# Autodesk Inventor assembly: ASY MSC 900.5 base frame
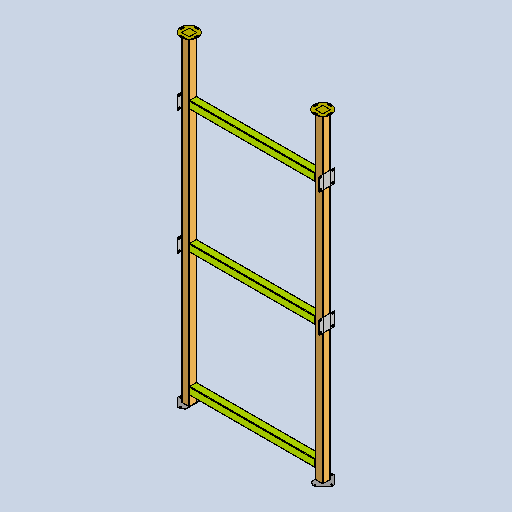
[picture p0: Inventor's stored thumbnail of the model, 512x512]
Saved by Autodesk Inventor 2025 (Build 290162010, 162A)
## iProperties
_SolveAssemblyDoc: Frame Generator Solve Assembly
_Version: 25.0.0
Created: 2024-06-27
Part Number: ASY MSC 900.5 base frame
Document SubType Name: Assembly
Designer: admin
Stock Number: ASY МОО 900.5 базовая рама
Author: admin
## Documents named in this file (7)
- C:\Users\pokla\Documents\Inventor\Отстойник осветлитель\Manturovo_Se-clar-Gleb\Pillars\ASY MSC 900.5 base frame.iam
- C:\Users\pokla\Documents\Inventor\Отстойник осветлитель\Manturovo_Se-clar-Gleb\MSC DIM 009.5 base frame sketch.ipt
- C:\Users\pokla\Documents\Inventor\Отстойник осветлитель\Manturovo_Se-clar-Gleb\Pillars\ASY MSC 900.5.1 base frame.iam
- C:\Users\pokla\Documents\Inventor\Отстойник осветлитель\Manturovo_Se-clar-Gleb\MSC DIM 001 frame.ipt
- C:\Users\pokla\Documents\Inventor\Отстойник осветлитель\Manturovo_Se-clar-Gleb\MSC 902 flange frame heel.ipt
- C:\Users\pokla\Documents\Inventor\Отстойник осветлитель\Manturovo_Se-clar-Gleb\MSC 906 flange frame.ipt
- C:\Users\pokla\Documents\Inventor\Отстойник осветлитель\Manturovo_Se-clar-Gleb\MSC 908 transverse pillar plate.ipt
## Components (10 placed, 5 different names)
1. MSC DIM 009.5 base frame sketch.ipt:1 — Mate:1, Flush:1, Flush:2
2. ASY MSC 900.5.1 base frame.iam:1 [sub-assembly] — Rigid:3, Rigid:4, Rigid:5, Rigid:6, Rigid:7, Rigid:8, Rigid:9, Rigid:10
3. MSC 902 flange frame heel.ipt:1 — Rigid:5
4. MSC 902 flange frame heel.ipt:2 — Rigid:6
5. MSC 906 flange frame.ipt:1 — Rigid:3
6. MSC 906 flange frame.ipt:2 — Rigid:4
7. MSC 908 transverse pillar plate.ipt:1 — Rigid:7
8. MSC 908 transverse pillar plate.ipt:2 — Rigid:8
9. MSC 908 transverse pillar plate.ipt:3 — Rigid:9
10. MSC 908 transverse pillar plate.ipt:4 — Rigid:10
## Relationships (11: WeldJoint 8, Flush 2, Mate 1)
- Rigid:3 [WeldJoint]: ASY MSC 900.5.1 base frame.iam:1 ↔ MSC 906 flange frame.ipt:1
- Rigid:4 [WeldJoint]: ASY MSC 900.5.1 base frame.iam:1 ↔ MSC 906 flange frame.ipt:2
- Rigid:5 [WeldJoint]: ASY MSC 900.5.1 base frame.iam:1 ↔ MSC 902 flange frame heel.ipt:1
- Rigid:6 [WeldJoint]: ASY MSC 900.5.1 base frame.iam:1 ↔ MSC 902 flange frame heel.ipt:2
- Mate:1: MSC DIM 009.5 base frame sketch.ipt:1
- Flush:1: MSC DIM 009.5 base frame sketch.ipt:1
- Flush:2: MSC DIM 009.5 base frame sketch.ipt:1
- Rigid:7 [WeldJoint] (80 mm): ASY MSC 900.5.1 base frame.iam:1 ↔ MSC 908 transverse pillar plate.ipt:1
- Rigid:8 [WeldJoint] (80 mm): ASY MSC 900.5.1 base frame.iam:1 ↔ MSC 908 transverse pillar plate.ipt:2
- Rigid:9 [WeldJoint] (80 mm): ASY MSC 900.5.1 base frame.iam:1 ↔ MSC 908 transverse pillar plate.ipt:3
- Rigid:10 [WeldJoint] (80 mm): ASY MSC 900.5.1 base frame.iam:1 ↔ MSC 908 transverse pillar plate.ipt:4
## Named parameters: frame_1 = 334.24956 mm, frame_3 = 2905.4 mm, frame_4 = 4190.97522 mm, frame_5 = 5476.55043 mm, Ширина_рамы = 1450 mm, Отступ_до_ниж_перекладины = 100 mm, Отступ_до_сред_перекладины = 1450 mm, Шаг_опор_по_баку = 2000 mm, Движение_рамы_вперед_назад = 270 mm, frame_2 = 1619.82478 mm, frame_6 = 6762.12565 mm, Высота_опорных_стоек = 151 mm
